# Autodesk Inventor assembly: Sprocket
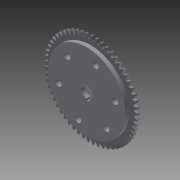
[picture p0: Inventor's stored thumbnail of the model, 180x180]
Saved by Autodesk Inventor 2013 (Build 170138000, 138)
## iProperties
Created: 2013-01-31
Part Number: Sprocket
Document SubType Name: Assembly
Designer: aslane
Author: aslane
## Documents named in this file (3)
- H:\Sprocket.iam
- H:\Arm Motor Assembly\Design Accelerator\Spur Gear21.ipt
- H:\Fitting piece for Sprocket.ipt
## Components (2 placed, 2 different names)
1. Spur Gear2:1 — Mate:1, Mate:2, Insert:1, Mate:3
2. Fitting piece for Sprocket:1 — Mate:1, Mate:2, Insert:1, Mate:3
## Relationships (4: Mate 3, Insert 1)
- Mate:1: Spur Gear2:1 ↔ Fitting piece for Sprocket:1
- Mate:2: Spur Gear2:1 ↔ Fitting piece for Sprocket:1
- Insert:1: Spur Gear2:1 ↔ Fitting piece for Sprocket:1
- Mate:3 (23.7871 mm): Spur Gear2:1 ↔ Fitting piece for Sprocket:1
